# Autodesk Inventor assembly: Claw
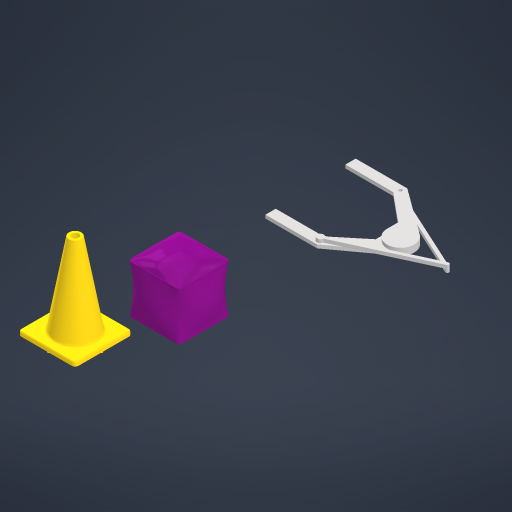
[picture p0: Inventor's stored thumbnail of the model, 512x512]
Saved by Autodesk Inventor 2023 (Build 270158000, 158)
## iProperties
Created: 2023-01-16
Part Number: Claw
Document SubType Name: Assembly
Designer: Terrence
Author: Terrence
## Documents named in this file (7)
- C:\Users\Terrence\Documents\FRC Long\Claw.iam
- C:\Users\Terrence\Documents\FRC Long\Solid1.ipt
- C:\Users\Terrence\Documents\FRC Long\Solid4.ipt
- C:\Users\Terrence\Documents\FRC Long\Solid2.ipt
- C:\Users\Terrence\Documents\FRC Long\Solid3.ipt
- C:\Users\Terrence\Downloads\GE-23700-Cone-STEP\GE-23700.ipt
- C:\Users\Terrence\Downloads\GE-23701-Cube-STEP\GE-23701.ipt
## Components (6 placed, 6 different names)
1. Solid1:1 — Insert:1, Insert:3
2. Solid4:1 — Insert:2, Insert:4
3. Solid2:1 — Insert:1, Insert:2
4. Solid3:1 — Insert:3, Insert:4
5. GE-23700:1
6. GE-23701:1
## Relationships (4: Insert 4)
- Insert:1: Solid1:1 ↔ Solid2:1
- Insert:2: Solid4:1 ↔ Solid2:1
- Insert:3: Solid1:1 ↔ Solid3:1
- Insert:4: Solid4:1 ↔ Solid3:1
